# Autodesk Inventor assembly: Tractive PCB
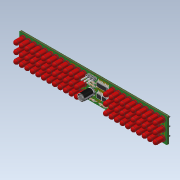
[picture p0: Inventor's stored thumbnail of the model, 180x180]
Saved by Autodesk Inventor 2021 (Build 250183000, 183)
## iProperties
Created: 2020-10-01
Part Number: Tractive PCB
Document SubType Name: Assembly
Designer: Administrator
Title: Tractive PCB v2
Author: Administrator
## Documents named in this file (8)
- C:\Users\capta\OneDrive - Lehigh University\Formula SAE\Tractive Light\PCB Assembly\Tractive PCB.iam
- C:\Users\capta\OneDrive - Lehigh University\Formula SAE\Tractive Light\PCB Assembly\Board.ipt
- C:\Users\capta\OneDrive - Lehigh University\Formula SAE\Tractive Light\PCB Assembly\Packages.iam
- C:\Users\capta\OneDrive - Lehigh University\Formula SAE\Tractive Light\PCB Assembly\1-copper.ipt
- C:\Users\capta\OneDrive - Lehigh University\Formula SAE\Tractive Light\PCB Assembly\16-copper.ipt
- C:\Users\capta\OneDrive - Lehigh University\Formula SAE\Tractive Light\PCB Assembly\1-soldermask.ipt
- C:\Users\capta\OneDrive - Lehigh University\Formula SAE\Tractive Light\PCB Assembly\16-soldermask.ipt
- C:\Users\capta\OneDrive - Lehigh University\Formula SAE\Tractive Light\Caps\Aluminum_electrolytic_capacitor_radial_D6.3_H11_PinD0.5_Pitch2.5_nominal_black_TOP.iam
## Components (7 placed, 7 different names)
1. Board:1
2. Packages:1 [sub-assembly]
3. 1-copper:1 — Mate:1
4. 16-copper:1
5. 1-soldermask:1
6. 16-soldermask:1
7. Aluminum_electrolytic_capacitor_radial_D6.3_H11_PinD0.5_Pitch2.5_nominal_black_TOP:1 [sub-assembly] — Mate:1
## Relationships (1: Mate 1)
- Mate:1: 1-copper:1 ↔ Aluminum_electrolytic_capacitor_radial_D6.3_H11_PinD0.5_Pitch2.5_nominal_black_TOP:1
